# Autodesk Inventor assembly: 000.007 - Куб типа Ш (красный)
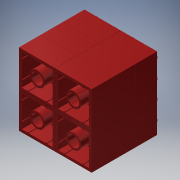
[picture p0: Inventor's stored thumbnail of the model, 180x180]
Saved by Autodesk Inventor 2019 (Build 230136000, 136)
## iProperties
Created: 2020-02-29
Part Number: 000.007 - Куб типа Ш (красный)
Material: Типовые
Document SubType Name: Assembly
Designer: Петров Иван
Author: Петров Иван
## Documents named in this file (2)
- E:\IVAN\Ivan_desktop\GitHub\Manipulation_IRS\hardware\000.007 - Куб типа Ш (красный).iam
- E:\IVAN\Ivan_desktop\GitHub\Manipulation_IRS\hardware\components\modular-lego-brick-standard-1.snapshot.7\Brick standard 4x2.ipt
## Components (6 placed, 1 different names)
1. Brick standard 4x2:2 — Совмещение:1, Заподлицо:1, Заподлицо:2
2. Brick standard 4x2:1 — Совмещение:1, Заподлицо:1, Заподлицо:2
3. Brick standard 4x2:3
4. Brick standard 4x2:4
5. Brick standard 4x2:5
6. Brick standard 4x2:6
## Component patterns: (3 elements, first: Brick standard 4x2:2 + Brick standard 4x2:1)
## Relationships (3: Flush 2, Mate 1)
- Совмещение:1 [Mate]: Brick standard 4x2:2 ↔ Brick standard 4x2:1
- Заподлицо:1 [Flush]: Brick standard 4x2:2 ↔ Brick standard 4x2:1
- Заподлицо:2 [Flush]: Brick standard 4x2:2 ↔ Brick standard 4x2:1
